# Autodesk Inventor assembly: рука
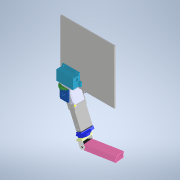
[picture p0: Inventor's stored thumbnail of the model, 180x180]
Saved by Autodesk Inventor 2022 (Build 260153000, 153)
## iProperties
Created: 2022-12-04
Part Number: рука
Document SubType Name: Assembly
Designer: Папа
Author: Папа
## Documents named in this file (11)
- F:\Новая папка\рука.iam
- F:\Новая папка\мотор_плеча_2.ipt
- F:\Новая папка\мотор_плеча_2.1-локтя_1.ipt
- F:\Новая папка\Servo body.ipt
- F:\Новая папка\мотор_локтя_2.1-кисти_1.ipt
- F:\Новая папка\servoDS3115mg.iam
- F:\Новая папка\мотор_локтя_1.1.ipt
- F:\Новая папка\подш.ipt
- F:\Новая папка\Сборка1.iam
- F:\Новая папка\Сборка7.iam
- F:\Новая папка\rds3115mg-servo-1.snapshot.1\RDS3115MG Servo.iam
## Components (11 placed, 10 different names)
1. мотор_плеча_2.1-локтя_1:1 — Совмещение:9, Совмещение:10, Совмещение:11, Совмещение:12, Совмещение:25, Совмещение:26, Совмещение:27, Совмещение:31
2. Servo body:1 — Совмещение:9, Совмещение:10, Совмещение:11, Совмещение:12, Совмещение:30
3. мотор_локтя_2.1-кисти_1:1 — Совмещение:54, Совмещение:55, Совмещение:56
4. servoDS3115mg:1 [sub-assembly] — Совмещение:25, Совмещение:26, Совмещение:27, Совмещение:32, Совмещение:33, Совмещение:34, Совмещение:47, Совмещение:48
5. мотор_плеча_2:1 — Совмещение:30, Совмещение:31, Совмещение:42, Совмещение:43, Совмещение:44, Совмещение:45
6. мотор_локтя_1.1:1 — Совмещение:32, Совмещение:33, Совмещение:34, Совмещение:46, Совмещение:47, Совмещение:48, Совмещение:49
7. подш:2 — Совмещение:42
8. Сборка1:1 [sub-assembly] — Совмещение:43, Совмещение:44, Совмещение:45
9. Сборка7:1 [sub-assembly] — Совмещение:50, Совмещение:51, Совмещение:52, Совмещение:53
10. подш:3 — Совмещение:46, Совмещение:49, Совмещение:50, Совмещение:51
11. RDS3115MG Servo:1 [sub-assembly] — Совмещение:52, Совмещение:53, Совмещение:54, Совмещение:55, Совмещение:56
## Relationships (27: Mate 27)
- Совмещение:9 [Mate]: мотор_плеча_2.1-локтя_1:1 ↔ Servo body:1
- Совмещение:10 [Mate]: мотор_плеча_2.1-локтя_1:1 ↔ Servo body:1
- Совмещение:11 [Mate]: мотор_плеча_2.1-локтя_1:1 ↔ Servo body:1
- Совмещение:12 [Mate]: мотор_плеча_2.1-локтя_1:1 ↔ Servo body:1
- Совмещение:25 [Mate]: мотор_плеча_2.1-локтя_1:1 ↔ servoDS3115mg:1
- Совмещение:26 [Mate]: мотор_плеча_2.1-локтя_1:1 ↔ servoDS3115mg:1
- Совмещение:27 [Mate]: мотор_плеча_2.1-локтя_1:1 ↔ servoDS3115mg:1
- Совмещение:30 [Mate]: Servo body:1 ↔ мотор_плеча_2:1
- Совмещение:31 [Mate]: мотор_плеча_2.1-локтя_1:1 ↔ мотор_плеча_2:1
- Совмещение:32 [Mate]: servoDS3115mg:1 ↔ мотор_локтя_1.1:1
- Совмещение:33 [Mate]: servoDS3115mg:1 ↔ мотор_локтя_1.1:1
- Совмещение:34 [Mate]: servoDS3115mg:1 ↔ мотор_локтя_1.1:1
- Совмещение:42 [Mate]: мотор_плеча_2:1 ↔ подш:2
- Совмещение:43 [Mate]: мотор_плеча_2:1 ↔ Сборка1:1
- Совмещение:44 [Mate]: мотор_плеча_2:1 ↔ Сборка1:1
- Совмещение:45 [Mate]: мотор_плеча_2:1 ↔ Сборка1:1
- Совмещение:46 [Mate]: мотор_локтя_1.1:1 ↔ подш:3
- Совмещение:47 [Mate]: servoDS3115mg:1 ↔ мотор_локтя_1.1:1
- Совмещение:48 [Mate]: servoDS3115mg:1 ↔ мотор_локтя_1.1:1
- Совмещение:49 [Mate]: мотор_локтя_1.1:1 ↔ подш:3
- Совмещение:50 [Mate]: Сборка7:1 ↔ подш:3
- Совмещение:51 [Mate]: Сборка7:1 ↔ подш:3
- Совмещение:52 [Mate]: Сборка7:1 ↔ RDS3115MG Servo:1
- Совмещение:53 [Mate] (0.05 mm): Сборка7:1 ↔ RDS3115MG Servo:1
- Совмещение:54 [Mate]: мотор_локтя_2.1-кисти_1:1 ↔ RDS3115MG Servo:1
- Совмещение:55 [Mate]: мотор_локтя_2.1-кисти_1:1 ↔ RDS3115MG Servo:1
- Совмещение:56 [Mate]: мотор_локтя_2.1-кисти_1:1 ↔ RDS3115MG Servo:1
